# Autodesk Inventor assembly: Gesamt
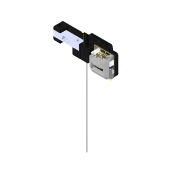
[picture p0: Inventor's stored thumbnail of the model, 180x180]
Saved by Autodesk Inventor 2022.3 (Build 263350000, 350)
## iProperties
Created: 2021-05-08
Part Number: Gesamt
Document SubType Name: Assembly
Designer: Sven
Author: Sven
## Documents named in this file (8)
- C:\Users\SUPPELT\Desktop\MesstechnikPraktikumV6\hardware\Endeffektor\cad\Gesamt.iam
- C:\Users\SUPPELT\Desktop\MesstechnikPraktikumV6\hardware\Endeffektor\cad\micro load cell CZL635.ipt
- C:\Users\SUPPELT\Desktop\MesstechnikPraktikumV6\hardware\Endeffektor\cad\Flansch_Simple.ipt
- C:\Users\SUPPELT\Desktop\MesstechnikPraktikumV6\hardware\Endeffektor\cad\NadelHalterLose.ipt
- C:\Users\SUPPELT\Desktop\MesstechnikPraktikumV6\hardware\Endeffektor\cad\NadelhalterSchraub.ipt
- C:\Users\SUPPELT\Desktop\MesstechnikPraktikumV6\hardware\Endeffektor\cad\Nadel.ipt
- C:\Users\SUPPELT\Desktop\MesstechnikPraktikumV6\hardware\Endeffektor\cad\42mm_Erweiterungsplatine v2.ipt
- C:\Users\SUPPELT\Desktop\MesstechnikPraktikumV6\hardware\Endeffektor\cad\SensorPlatineAbdeckung.ipt
## Components (7 placed, 7 different names)
1. Flansch_Simple:1 — Passend:14, Passend:19, Fluchtend:3, Fluchtend:4, Fluchtend:5, Fluchtend:6
2. micro load cell CZL635:1 — Passend:8, Passend:9, Passend:10
3. NadelHalterLose:1 — Passend:11, Fluchtend:1, Fluchtend:2, Passend:14, Passend:17, Passend:18, Winkel:1
4. NadelhalterSchraub:1 — Passend:8, Passend:9, Passend:10, Passend:11, Fluchtend:1, Fluchtend:2
5. Nadel:1 — Passend:17, Passend:18, Winkel:1
6. 42mm_Erweiterungsplatine v2:1 — Passend:19, Fluchtend:3, Fluchtend:4, Passend:20
7. SensorPlatineAbdeckung:1 — Passend:20, Fluchtend:5, Fluchtend:6
## Relationships (16: Mate 9, Flush 6, Angle 1)
- Passend:8 [Mate]: micro load cell CZL635:1 ↔ NadelhalterSchraub:1
- Passend:9 [Mate]: micro load cell CZL635:1 ↔ NadelhalterSchraub:1
- Passend:10 [Mate]: micro load cell CZL635:1 ↔ NadelhalterSchraub:1
- Passend:11 [Mate]: NadelHalterLose:1 ↔ NadelhalterSchraub:1
- Fluchtend:1 [Flush]: NadelHalterLose:1 ↔ NadelhalterSchraub:1
- Fluchtend:2 [Flush]: NadelHalterLose:1 ↔ NadelhalterSchraub:1
- Passend:14 [Mate] (1.25 mm): Flansch_Simple:1 ↔ NadelHalterLose:1
- Passend:17 [Mate]: NadelHalterLose:1 ↔ Nadel:1
- Passend:18 [Mate]: NadelHalterLose:1 ↔ Nadel:1
- Winkel:1 [Angle] (0 deg): NadelHalterLose:1 ↔ Nadel:1
- Passend:19 [Mate]: Flansch_Simple:1 ↔ 42mm_Erweiterungsplatine v2:1
- Fluchtend:3 [Flush]: Flansch_Simple:1 ↔ 42mm_Erweiterungsplatine v2:1
- Fluchtend:4 [Flush]: Flansch_Simple:1 ↔ 42mm_Erweiterungsplatine v2:1
- Passend:20 [Mate]: 42mm_Erweiterungsplatine v2:1 ↔ SensorPlatineAbdeckung:1
- Fluchtend:5 [Flush]: Flansch_Simple:1 ↔ SensorPlatineAbdeckung:1
- Fluchtend:6 [Flush]: Flansch_Simple:1 ↔ SensorPlatineAbdeckung:1
